# Autodesk Inventor assembly: Door Assembly
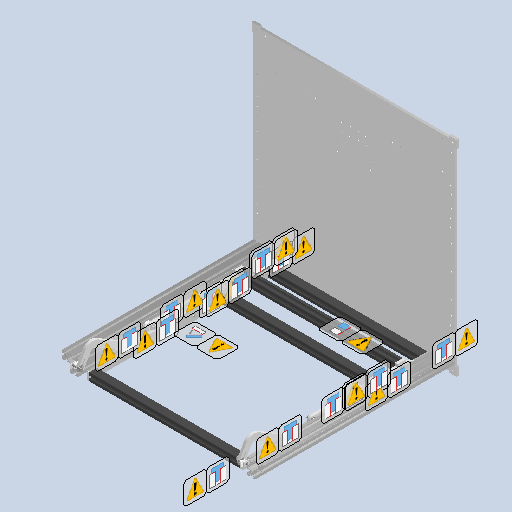
[picture p0: Inventor's stored thumbnail of the model, 512x512]
Saved by Autodesk Inventor 2024 (Build 280153000, 153)
## iProperties
Created: 2024-08-28
Part Number: Door Assembly
Document SubType Name: Assembly
Designer: Ishaan
Author: Ishaan
## Documents named in this file (16)
- E:\Projects\Axiom--IDEX-3D-Printer\CAD\06 - Door\Door Assembly.iam
- E:\Projects\Axiom--IDEX-3D-Printer\CAD\06 - Door\Door Aluminum Bars.ipt
- E:\Projects\Axiom--IDEX-3D-Printer\CAD\02 - Frame\Printer Base Plate RevI.ipt
- E:\Projects\Axiom--IDEX-3D-Printer\CAD\06 - Door\Door Lower Parallel Bar.ipt
- E:\Projects\Axiom--IDEX-3D-Printer\CAD\06 - Door\Door Upper Parallel Bar.ipt
- E:\Projects\Axiom--IDEX-3D-Printer\CAD\00 - COTS Components\F685ZZ.ipt
- E:\Projects\Axiom--IDEX-3D-Printer\CAD\06 - Door\Door Bar Bearing Spacer.ipt
- E:\Projects\Axiom--IDEX-3D-Printer\CAD\06 - Door\Door Bar Bearing Door Mounting Spacer.ipt
- E:\Projects\Axiom--IDEX-3D-Printer\CAD\00 - COTS Components\2020 Door Runners\HFSFB5-2020-375.ipt
- E:\Projects\Axiom--IDEX-3D-Printer\CAD\06 - Door\Door Bar Bearing Frame Mounting Spacer.ipt
- E:\Projects\Axiom--IDEX-3D-Printer\CAD\00 - COTS Components\2020 Door Bar Extrusion\HFSFB5-2020-393.ipt
- E:\Projects\Axiom--IDEX-3D-Printer\CAD\06 - Door\Door Panel.ipt
- E:\Projects\Axiom--IDEX-3D-Printer\CAD\00 - COTS Components\Hardware\SHCSM5x20.ipt
- E:\Projects\Axiom--IDEX-3D-Printer\CAD\00 - COTS Components\Hardware\M5 T SLOT NUT.ipt
- E:\Projects\Axiom--IDEX-3D-Printer\CAD\00 - COTS Components\Hardware\SHCSM5x16.ipt
- E:\Projects\Axiom--IDEX-3D-Printer\CAD\00 - COTS Components\4040 Vertical L Extrusions\HFS5-404020-475-SC.ipt
## Components (66 placed, 15 different names)
1. Door Aluminum Bars:1 — Insert:18, Insert:47
2. HFSFB5-2020-375:1
3. HFSFB5-2020-375:2
4. HFSFB5-2020-375:3 — Mate:10
5. Door Aluminum Bars:2 — Insert:26, Insert:48
6. Printer Base Plate RevI:1 — Mate:7, Mate:8
7. HFS5-404020-475-SC:1
8. HFS5-404020-475-SC:2
9. Door Lower Parallel Bar:1 — Insert:11, Insert:12, Insert:15, Insert:16, Insert:33
10. Door Upper Parallel Bar:1 — Insert:37, Insert:38, Insert:39, Insert:40
11. Door Bar Bearing Spacer:1 — Insert:14
12. Door Bar Bearing Spacer:2 — Insert:13
13. Door Bar Bearing Door Mounting Spacer:1 — Insert:17, Insert:18
14. Door Lower Parallel Bar:2 — Insert:19, Insert:20, Insert:23, Insert:24, Insert:34, Flush:8
15. Door Bar Bearing Spacer:3 — Insert:21
16. Door Bar Bearing Spacer:4 — Insert:22
17. Door Bar Bearing Door Mounting Spacer:2 — Insert:25, Insert:26
18. Door Bar Bearing Frame Mounting Spacer:1 — Insert:31, Mate:7, Flush:12
19. Door Bar Bearing Frame Mounting Spacer:2 — Insert:32, Mate:8, Flush:10
20. HFSFB5-2020-393:1 — Insert:33, Insert:34, Flush:8
21. Door Upper Parallel Bar:2 — Insert:43, Insert:44, Insert:45, Insert:46
22. Door Bar Bearing Spacer:5
23. Door Bar Bearing Spacer:6
24. Door Bar Bearing Spacer:7
25. Door Bar Bearing Spacer:8
26. Door Bar Bearing Door Mounting Spacer:3 — Insert:47, Insert:49
27. Door Bar Bearing Door Mounting Spacer:4 — Insert:48, Insert:50
28. Door Bar Bearing Frame Mounting Spacer:3 — Insert:51, Flush:10
29. Door Bar Bearing Frame Mounting Spacer:4 — Insert:52, Flush:12
30. Door Panel:1 — Mate:10
31. SHCSM5x16:1
32. SHCSM5x16:2
33. SHCSM5x16:3
34. SHCSM5x16:4
35. SHCSM5x16:5
36. SHCSM5x16:6
37. SHCSM5x16:7
38. SHCSM5x16:8
39. SHCSM5x16:9
40. SHCSM5x16:10
41. SHCSM5x16:11
42. SHCSM5x16:12
43. SHCSM5x20:1 — Insert:53, Mate:15
44. SHCSM5x20:2 — Insert:54, Mate:17
45. SHCSM5x20:3 — Insert:55, Mate:11
46. SHCSM5x20:4 — Insert:56, Mate:13
47. M5 T SLOT NUT:1 — Mate:15
48. M5 T SLOT NUT:2 — Mate:17
49. M5 T SLOT NUT:3 — Mate:13
50. M5 T SLOT NUT:4 — Mate:11
51. F685ZZ:5 — Insert:19, Insert:21
52. F685ZZ:6 — Insert:20, Insert:22, Insert:32
53. F685ZZ:7 — Insert:23, Insert:25
54. F685ZZ:8 — Insert:24, Insert:54
55. F685ZZ:1 — Insert:11, Insert:14, Insert:17
56. F685ZZ:2 — Insert:12, Insert:13, Insert:56
57. F685ZZ:3 — Insert:15
58. F685ZZ:4 — Insert:16, Insert:31
59. F685ZZ:13 — Insert:46
60. F685ZZ:14 — Insert:44, Insert:51
61. F685ZZ:15 — Insert:45, Insert:50
62. F685ZZ:16 — Insert:43, Insert:53
63. F685ZZ:9 — Insert:39, Insert:49
64. F685ZZ:10 — Insert:37, Insert:55
65. F685ZZ:11 — Insert:40
66. F685ZZ:12 — Insert:38, Insert:52
## Relationships (95: Insert 64, Mate 15, Flush 11, Angle 5)
- [Insert]: Door Aluminum Bars:1 ↔ HFSFB5-2020-375:2
- [Flush]: Door Aluminum Bars:1 ↔ HFSFB5-2020-375:2
- [Insert]: Door Aluminum Bars:1 ↔ HFSFB5-2020-375:3
- [Flush]: Door Aluminum Bars:1 ↔ HFSFB5-2020-375:3
- [Insert]: Door Aluminum Bars:1 ↔ HFSFB5-2020-375:1
- [Flush]: Door Aluminum Bars:1 ↔ HFSFB5-2020-375:1
- [Insert]: HFSFB5-2020-375:1 ↔ Door Aluminum Bars:2
- [Insert]: HFSFB5-2020-375:3 ↔ Door Aluminum Bars:2
- [Insert]: HFSFB5-2020-375:2 ↔ Door Aluminum Bars:2
- [Insert]: Printer Base Plate RevI:1 ↔ HFS5-404020-475-SC:1
- [Insert]: Printer Base Plate RevI:1 ↔ HFS5-404020-475-SC:1
- [Insert]: Printer Base Plate RevI:1 ↔ HFS5-404020-475-SC:2
- [Insert]: Printer Base Plate RevI:1 ↔ HFS5-404020-475-SC:2
- [Mate] (10 mm): HFSFB5-2020-375:2 ↔ Printer Base Plate RevI:1
- [Flush]: Door Aluminum Bars:1 ↔ HFS5-404020-475-SC:1
- Insert:11: Door Lower Parallel Bar:1 ↔ F685ZZ:1
- Insert:12: Door Lower Parallel Bar:1 ↔ F685ZZ:2
- Insert:13: Door Bar Bearing Spacer:2 ↔ F685ZZ:2
- Insert:14: Door Bar Bearing Spacer:1 ↔ F685ZZ:1
- Insert:15: Door Lower Parallel Bar:1 ↔ F685ZZ:3
- Insert:16: Door Lower Parallel Bar:1 ↔ F685ZZ:4
- Insert:17: Door Bar Bearing Door Mounting Spacer:1 ↔ F685ZZ:1
- Insert:18: Door Aluminum Bars:1 ↔ Door Bar Bearing Door Mounting Spacer:1
- Insert:19: Door Lower Parallel Bar:2 ↔ F685ZZ:5
- Insert:20: Door Lower Parallel Bar:2 ↔ F685ZZ:6
- Insert:21: Door Bar Bearing Spacer:3 ↔ F685ZZ:5
- Insert:22: Door Bar Bearing Spacer:4 ↔ F685ZZ:6
- Insert:23: Door Lower Parallel Bar:2 ↔ F685ZZ:7
- Insert:24: Door Lower Parallel Bar:2 ↔ F685ZZ:8
- Insert:25: Door Bar Bearing Door Mounting Spacer:2 ↔ F685ZZ:7
- Insert:26: Door Aluminum Bars:2 ↔ Door Bar Bearing Door Mounting Spacer:2
- Insert:31: Door Bar Bearing Frame Mounting Spacer:1 ↔ F685ZZ:4
- Insert:32: Door Bar Bearing Frame Mounting Spacer:2 ↔ F685ZZ:6
- [Mate]: HFS5-404020-475-SC:1 ↔ Door Bar Bearing Frame Mounting Spacer:1
- [Mate]: HFS5-404020-475-SC:2 ↔ Door Bar Bearing Frame Mounting Spacer:2
- [Flush] (4 mm): HFS5-404020-475-SC:2 ↔ Door Bar Bearing Frame Mounting Spacer:2
- [Flush] (4 mm): HFS5-404020-475-SC:1 ↔ Door Bar Bearing Frame Mounting Spacer:1
- Mate:7 (299 mm): Printer Base Plate RevI:1 ↔ Door Bar Bearing Frame Mounting Spacer:1
- Mate:8 (299 mm): Printer Base Plate RevI:1 ↔ Door Bar Bearing Frame Mounting Spacer:2
- [Angle] (0 deg): HFS5-404020-475-SC:1 ↔ Door Lower Parallel Bar:1
- Insert:33: Door Lower Parallel Bar:1 ↔ HFSFB5-2020-393:1
- Insert:34: Door Lower Parallel Bar:2 ↔ HFSFB5-2020-393:1
- Flush:8: Door Lower Parallel Bar:2 ↔ HFSFB5-2020-393:1
- [Insert]: Door Bar Bearing Spacer:5 ↔ F685ZZ:9
- [Insert]: Door Bar Bearing Spacer:6 ↔ F685ZZ:10
- Insert:37: Door Upper Parallel Bar:1 ↔ F685ZZ:10
- Insert:38: Door Upper Parallel Bar:1 ↔ F685ZZ:12
- Insert:39: Door Upper Parallel Bar:1 ↔ F685ZZ:9
- Insert:40: Door Upper Parallel Bar:1 ↔ F685ZZ:11
- [Insert]: Door Bar Bearing Spacer:7 ↔ F685ZZ:13
- [Insert]: Door Bar Bearing Spacer:8 ↔ F685ZZ:14
- Insert:43: Door Upper Parallel Bar:2 ↔ F685ZZ:16
- Insert:44: Door Upper Parallel Bar:2 ↔ F685ZZ:14
- Insert:45: Door Upper Parallel Bar:2 ↔ F685ZZ:15
- Insert:46: Door Upper Parallel Bar:2 ↔ F685ZZ:13
- Insert:47: Door Aluminum Bars:1 ↔ Door Bar Bearing Door Mounting Spacer:3
- Insert:48: Door Aluminum Bars:2 ↔ Door Bar Bearing Door Mounting Spacer:4
- Insert:49: Door Bar Bearing Door Mounting Spacer:3 ↔ F685ZZ:9
- Insert:50: Door Bar Bearing Door Mounting Spacer:4 ↔ F685ZZ:15
- Insert:51: Door Bar Bearing Frame Mounting Spacer:3 ↔ F685ZZ:14
- [Mate]: HFS5-404020-475-SC:2 ↔ Door Bar Bearing Frame Mounting Spacer:3
- [Flush] (-4 mm): HFS5-404020-475-SC:2 ↔ Door Bar Bearing Frame Mounting Spacer:3
- Flush:10 (-180 mm): Door Bar Bearing Frame Mounting Spacer:2 ↔ Door Bar Bearing Frame Mounting Spacer:3
- Insert:52: Door Bar Bearing Frame Mounting Spacer:4 ↔ F685ZZ:12
- [Flush] (4 mm): HFS5-404020-475-SC:1 ↔ Door Bar Bearing Frame Mounting Spacer:4
- Flush:12 (180 mm): Door Bar Bearing Frame Mounting Spacer:1 ↔ Door Bar Bearing Frame Mounting Spacer:4
- Mate:10: HFSFB5-2020-375:3 ↔ Door Panel:1
- Insert:53: SHCSM5x20:1 ↔ F685ZZ:16
- Insert:54: SHCSM5x20:2 ↔ F685ZZ:8
- Insert:55: SHCSM5x20:3 ↔ F685ZZ:10
- Insert:56: SHCSM5x20:4 ↔ F685ZZ:2
- Mate:11: SHCSM5x20:3 ↔ M5 T SLOT NUT:4
- [Mate]: HFS5-404020-475-SC:1 ↔ M5 T SLOT NUT:4
- [Angle] (0 deg): HFS5-404020-475-SC:1 ↔ M5 T SLOT NUT:4
- Mate:13: SHCSM5x20:4 ↔ M5 T SLOT NUT:3
- [Mate]: HFS5-404020-475-SC:1 ↔ M5 T SLOT NUT:3
- [Angle] (0 deg): HFS5-404020-475-SC:1 ↔ M5 T SLOT NUT:3
- Mate:15: SHCSM5x20:1 ↔ M5 T SLOT NUT:1
- [Mate]: HFS5-404020-475-SC:2 ↔ M5 T SLOT NUT:1
- [Angle] (0 deg): HFS5-404020-475-SC:2 ↔ M5 T SLOT NUT:1
- Mate:17: SHCSM5x20:2 ↔ M5 T SLOT NUT:2
- [Mate]: HFS5-404020-475-SC:2 ↔ M5 T SLOT NUT:2
- [Angle] (0 deg): HFS5-404020-475-SC:2 ↔ M5 T SLOT NUT:2
- [Insert]: SHCSM5x16:1 ↔ F685ZZ:11
- [Insert]: SHCSM5x16:2 ↔ F685ZZ:3
- [Insert]: SHCSM5x16:3 ↔ F685ZZ:13
- [Insert]: SHCSM5x16:4 ↔ F685ZZ:5
- [Insert]: Door Aluminum Bars:1 ↔ SHCSM5x16:9
- [Insert]: Door Lower Parallel Bar:1 ↔ SHCSM5x16:10
- [Insert]: Door Aluminum Bars:1 ↔ SHCSM5x16:11
- [Insert]: Door Aluminum Bars:1 ↔ SHCSM5x16:12
- [Insert]: Door Aluminum Bars:2 ↔ SHCSM5x16:7
- [Insert]: Door Aluminum Bars:2 ↔ SHCSM5x16:8
- [Insert]: Door Lower Parallel Bar:2 ↔ SHCSM5x16:6
- [Insert]: Door Aluminum Bars:2 ↔ SHCSM5x16:5
## Named parameters: d70_d44 = 0 mm, d71_d45 = 0 mm, d76_d70_d44 = 0 mm, d77_d71_d45 = 0 mm
